# Autodesk Inventor assembly: BackStand
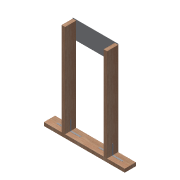
[picture p0: Inventor's stored thumbnail of the model, 180x180]
Saved by Autodesk Inventor 2017 (Build 210142000, 142)
## iProperties
Created: 2017-05-22
Part Number: BackStand
Document SubType Name: Assembly
Designer: krosie
Author: krosie
## Documents named in this file (6)
- C:\Users\krosie\Google Drive\HERA\hera-cad\Node\Fan\Mount\BackStand.iam
- FrontStand.iam
- C:\Users\krosie\Google Drive\HERA\hera-cad\Node\Fan\Mount\BaseStand.ipt
- C:\Users\krosie\Google Drive\HERA\hera-cad\Node\Fan\Mount\80mmCornerBracket.ipt
- C:\Users\krosie\Google Drive\HERA\hera-cad\Node\Fan\Mount\BackVerticalMount.ipt
- C:\Users\krosie\Google Drive\HERA\hera-cad\Node\Fan\Mount\MountVertical.ipt
## Components (8 placed, 4 different names)
1. BaseStand:1 — Mate:7, Mate:9, Flush:12, Flush:13, Mate:10, Mate:11, Flush:14, Flush:15, Flush:18, Mate:15, Mate:16
2. 30mmCornerBracket:1 — Mate:9, Flush:12, Mate:13, Flush:19
3. 30mmCornerBracket:4 — Mate:7, Flush:13, Mate:14, Flush:20
4. MountVertical:1 — Mate:10, Flush:14, Mate:12, Flush:16, Mate:14, Mate:17
5. MountVertical:2 — Mate:11, Flush:15, Flush:17, Flush:18, Mate:13, Mate:18
6. BackVerticalMount:1 — Mate:12, Flush:16, Flush:17
7. 30mmCornerBracket:5 — Mate:16, Mate:18, Flush:19
8. 30mmCornerBracket:6 — Mate:15, Mate:17, Flush:20
## Relationships (20: Mate 11, Flush 9)
- Mate:7: BaseStand:1 ↔ 30mmCornerBracket:4
- Mate:9: BaseStand:1 ↔ 30mmCornerBracket:1
- Flush:12 (47.5 mm): BaseStand:1 ↔ 30mmCornerBracket:1
- Flush:13 (47.5 mm): BaseStand:1 ↔ 30mmCornerBracket:4
- Mate:10: BaseStand:1 ↔ MountVertical:1
- Mate:11: BaseStand:1 ↔ MountVertical:2
- Flush:14: BaseStand:1 ↔ MountVertical:1
- Flush:15: BaseStand:1 ↔ MountVertical:2
- Mate:12: MountVertical:1 ↔ BackVerticalMount:1
- Flush:16: MountVertical:1 ↔ BackVerticalMount:1
- Flush:17: MountVertical:2 ↔ BackVerticalMount:1
- Flush:18 (175 mm): BaseStand:1 ↔ MountVertical:2
- Mate:13: 30mmCornerBracket:1 ↔ MountVertical:2
- Mate:14: 30mmCornerBracket:4 ↔ MountVertical:1
- Mate:15: BaseStand:1 ↔ 30mmCornerBracket:6
- Mate:16: BaseStand:1 ↔ 30mmCornerBracket:5
- Mate:17: MountVertical:1 ↔ 30mmCornerBracket:6
- Mate:18: MountVertical:2 ↔ 30mmCornerBracket:5
- Flush:19: 30mmCornerBracket:1 ↔ 30mmCornerBracket:5
- Flush:20: 30mmCornerBracket:4 ↔ 30mmCornerBracket:6
